# Autodesk Inventor assembly: 整车装配体
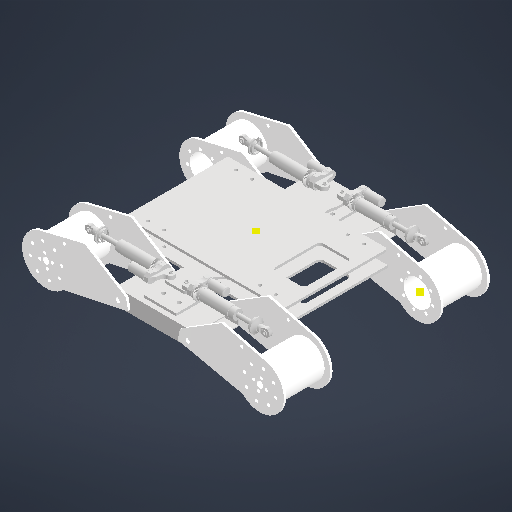
[picture p0: Inventor's stored thumbnail of the model, 512x512]
Saved by Autodesk Inventor 2025 (Build 290162000, 162)
## iProperties
Created: 2026-01-01
Part Number: 整车装配体
Document SubType Name: Assembly
Designer: XH
Author: XH
## Documents named in this file (13)
- D:\gitdesktop\THE_Car\模型库\整车装配体.iam
- D:\gitdesktop\THE_Car\模型库\电机装配.iam
- D:\gitdesktop\THE_Car\模型库\小车主体.ipt
- D:\gitdesktop\THE_Car\模型库\铝方管.ipt
- D:\gitdesktop\THE_Car\模型库\电机装配_MIR.iam
- D:\gitdesktop\THE_Car\模型库\电机装配_MIR1.iam
- D:\gitdesktop\THE_Car\模型库\铝方管_MIR.ipt
- D:\gitdesktop\THE_Car\模型库\电机装配_MIR_MIR.iam
- D:\gitdesktop\THE_Car\模型库\板子.ipt
- D:\gitdesktop\THE_Car\模型库\顶板装配隔离.ipt
- D:\gitdesktop\THE_Car\模型库\连杆1.ipt
- D:\gitdesktop\THE_Car\模型库\三角连杆.ipt
- D:\gitdesktop\THE_Car\模型库\KJ110FT33装配体.iam
## Components (16 placed, 12 different names)
1. 电机装配:1 [sub-assembly] — 配合:1, 配合:2, 配合:23
2. 小车主体:1
3. 铝方管:1 — 配合:1, 配合:2, 配合:3, 表面齐平:1, 配合:12
4. 电机装配_MIR:1 [sub-assembly] — 配合:3, 配合:8, 配合:11, 配合:12, 配合:27
5. 电机装配_MIR1:1 [sub-assembly] — 配合:4, 配合:5
6. 铝方管_MIR:1 — 配合:4, 配合:5, 配合:6, 配合:7, 表面齐平:1, 配合:9
7. 电机装配_MIR_MIR:1 [sub-assembly] — 配合:6, 配合:7, 配合:8, 配合:10, 配合:28
8. 板子:1 — 配合:9, 配合:10, 配合:11, 配合:13, 表面齐平:2, 配合:14, 配合:15, 配合:25, 配合:26
9. 顶板装配隔离:1 — 配合:13, 表面齐平:2, 配合:14
10. 连杆1:1 — 配合:15, 配合:16, 配合:18, 配合:22, 配合:24
11. 三角连杆:1 — 配合:16, 配合:18, 配合:20, 配合:26
12. KJ110FT33装配体:1 [sub-assembly] — 配合:20
13. 三角连杆:2 — 配合:22, 配合:24, 配合:25
14. KJ110FT33装配体:2 [sub-assembly] — 配合:23
15. KJ110FT33装配体:3 [sub-assembly] — 配合:27
16. KJ110FT33装配体:4 [sub-assembly] — 配合:28
## Relationships (27: Mate 25, Flush 2)
- 配合:1 [Mate]: 电机装配:1 ↔ 铝方管:1
- 配合:2 [Mate]: 电机装配:1 ↔ 铝方管:1
- 配合:3 [Mate]: 铝方管:1 ↔ 电机装配_MIR:1
- 配合:4 [Mate]: 电机装配_MIR1:1 ↔ 铝方管_MIR:1
- 配合:5 [Mate]: 电机装配_MIR1:1 ↔ 铝方管_MIR:1
- 配合:6 [Mate]: 铝方管_MIR:1 ↔ 电机装配_MIR_MIR:1
- 配合:7 [Mate]: 铝方管_MIR:1 ↔ 电机装配_MIR_MIR:1
- 表面齐平:1 [Flush]: 铝方管:1 ↔ 铝方管_MIR:1
- 配合:8 [Mate]: 电机装配_MIR:1 ↔ 电机装配_MIR_MIR:1
- 配合:9 [Mate]: 铝方管_MIR:1 ↔ 板子:1
- 配合:10 [Mate] (3 mm): 电机装配_MIR_MIR:1 ↔ 板子:1
- 配合:11 [Mate] (3 mm): 电机装配_MIR:1 ↔ 板子:1
- 配合:12 [Mate]: 铝方管:1 ↔ 电机装配_MIR:1
- 配合:13 [Mate] (15 mm): 板子:1 ↔ 顶板装配隔离:1
- 表面齐平:2 [Flush]: 板子:1 ↔ 顶板装配隔离:1
- 配合:14 [Mate]: 板子:1 ↔ 顶板装配隔离:1
- 配合:15 [Mate] (5 mm): 板子:1 ↔ 连杆1:1
- 配合:16 [Mate]: 连杆1:1 ↔ 三角连杆:1
- 配合:18 [Mate]: 连杆1:1 ↔ 三角连杆:1
- 配合:20 [Mate]: 三角连杆:1 ↔ KJ110FT33装配体:1
- 配合:22 [Mate]: 连杆1:1 ↔ 三角连杆:2
- 配合:23 [Mate]: 电机装配:1 ↔ KJ110FT33装配体:2
- 配合:24 [Mate]: 连杆1:1 ↔ 三角连杆:2
- 配合:25 [Mate]: 板子:1 ↔ 三角连杆:2
- 配合:26 [Mate]: 板子:1 ↔ 三角连杆:1
- 配合:27 [Mate]: 电机装配_MIR:1 ↔ KJ110FT33装配体:3
- 配合:28 [Mate]: 电机装配_MIR_MIR:1 ↔ KJ110FT33装配体:4
